# Autodesk Inventor assembly: 6001 BEARING
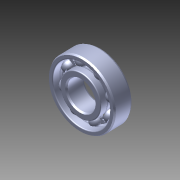
[picture p0: Inventor's stored thumbnail of the model, 180x180]
Saved by Autodesk Inventor 2015 (Build 190159000, 159)
## iProperties
Created: 2014-09-08
Part Number: 6001 BEARING
Document SubType Name: Assembly
Designer: laca
Mass: 2.58366 g
Surface Area: 37.5438 cm^2
Volume: 2.58366 cm^3
Density: 1 g/cm^3
Title: 6001 BEARING.STEP
Description: STEP AP214
Creation Date: 2014-04-05
Sending System: SolidWorks 2012
Preprocessor: SwSTEP 2.0
Author: laca
## Documents named in this file (5)
- C:\Users\laca\Desktop\iRoobo2014Ver3\6001 BEARING.iam
- C:\Users\laca\Desktop\iRoobo2014Ver3\6001 Outer.ipt
- C:\Users\laca\Desktop\iRoobo2014Ver3\6001 Inner.ipt
- C:\Users\laca\Desktop\iRoobo2014Ver3\6001 Guide.ipt
- C:\Users\laca\Desktop\iRoobo2014Ver3\6001 Ball.ipt
## Components (12 placed, 12 different names)
1. 6001 Outer_1 — Insert:1
2. 6001 Inner_2 — Insert:1, Insert:2
3. 6001 Guide_3 — Rigid:1, Insert:2, Ball:2, Ball:3, Ball:4, Ball:5, Ball:6, Ball:7, Ball:8
4. 6001 Guide_4 — Rigid:1, Ball:1
5. 6001 Ball_5 — Ball:6
6. 6001 Ball_6 — Ball:7
7. 6001 Ball_7 — Ball:8
8. 6001 Ball_8 — Ball:1
9. 6001 Ball_9 — Ball:2
10. 6001 Ball_10 — Ball:3
11. 6001 Ball_11 — Ball:4
12. 6001 Ball_12 — Ball:5
## Relationships (11: BallJoint 8, Insert 2, WeldJoint 1)
- Insert:1: 6001 Outer_1 ↔ 6001 Inner_2
- Rigid:1 [WeldJoint] (-0.5 mm): 6001 Guide_3 ↔ 6001 Guide_4
- Ball:1: 6001 Guide_4 ↔ 6001 Ball_8
- Insert:2 (-4 mm): 6001 Inner_2 ↔ 6001 Guide_3
- Ball:2: 6001 Guide_3 ↔ 6001 Ball_9
- Ball:3: 6001 Guide_3 ↔ 6001 Ball_10
- Ball:4: 6001 Guide_3 ↔ 6001 Ball_11
- Ball:5: 6001 Guide_3 ↔ 6001 Ball_12
- Ball:6: 6001 Guide_3 ↔ 6001 Ball_5
- Ball:7: 6001 Guide_3 ↔ 6001 Ball_6
- Ball:8: 6001 Guide_3 ↔ 6001 Ball_7
